# Autodesk Inventor assembly: A2017_T5_07
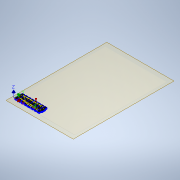
[picture p0: Inventor's stored thumbnail of the model, 180x180]
Saved by Autodesk Inventor 2020 (Build 240168000, 168)
## iProperties
Created: 2021-08-27
Part Number: A2017_T5_07
Document SubType Name: Assembly
Designer: Masato
Author: Masato
## Documents named in this file (3)
- D:\GitHub\inventor\SUSTAINA-OP\Cam\A2017_T5_07.iam
- D:\GitHub\inventor\SUSTAINA-OP\Cam\DisposableBoard.ipt
- D:\GitHub\inventor\SUSTAINA-OP\LowerBody\Foot\Foot_root_block.ipt
## Components (9 placed, 2 different names)
1. DisposableBoard:1 — メイト:2, メイト:1, フラッシュ:1, フラッシュ:2, メイト:4, メイト:5, メイト:6
2. Foot_root_block:1 — メイト:4, メイト:5, メイト:6
3. Foot_root_block:2
4. Foot_root_block:3
5. Foot_root_block:4
6. Foot_root_block:5
7. Foot_root_block:6
8. Foot_root_block:7
9. Foot_root_block:8
## Component patterns: (8 elements, first: Foot_root_block:1)
## Relationships (7: Mate 5, Flush 2)
- メイト:2 [Mate]: DisposableBoard:1
- メイト:1 [Mate]: DisposableBoard:1
- フラッシュ:1 [Flush]: DisposableBoard:1
- フラッシュ:2 [Flush]: DisposableBoard:1
- メイト:4 [Mate]: DisposableBoard:1 ↔ Foot_root_block:1
- メイト:5 [Mate] (2 mm): DisposableBoard:1 ↔ Foot_root_block:1
- メイト:6 [Mate] (2 mm): DisposableBoard:1 ↔ Foot_root_block:1
